# Autodesk Inventor assembly: SACMI DPA TILES GRIP
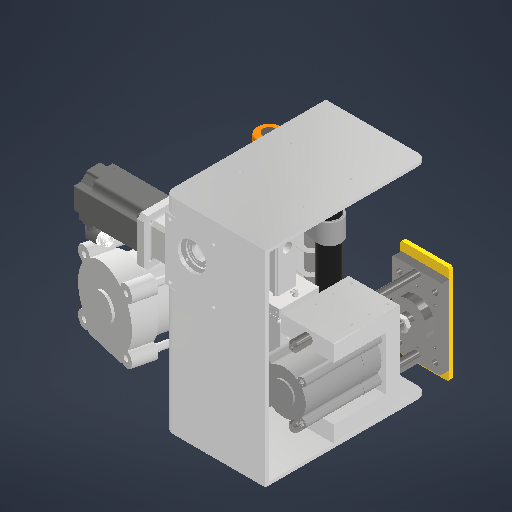
[picture p0: Inventor's stored thumbnail of the model, 512x512]
Saved by Autodesk Inventor 2025 (Build 290162000, 162)
## iProperties
Created: 2024-05-26
Part Number: SACMI DPA TILES GRIP
Document SubType Name: Assembly
Designer: zulet
Author: zulet
## Documents named in this file (7)
- D:\UNAL\2024-1S\APM\Digital Factory\Packaging Machine\SACMI DPA TILES GRIP_MIR.iam
- D:\UNAL\2024-1S\APM\Digital Factory\Linear Guides & Ball Screws\guidage_lineaire_shs55_lv_1_ss___492l_66.iam
- D:\UNAL\2024-1S\APM\Digital Factory\Packaging Machine\Assembly2.iam
- D:\UNAL\2024-1S\APM\Digital Factory\Packaging Machine\TILES GRIP ROLLERS.ipt
- D:\UNAL\2024-1S\APM\Digital Factory\Pneumatic Cylinders and Guides\cylinder_452500010050_010754_0.iam
- D:\UNAL\2024-1S\APM\Digital Factory\Pneumatic Cylinders and Guides\cylinder_45001223510555_0.iam
- D:\UNAL\2024-1S\APM\Digital Factory\Packaging Machine\SACMI DPA TILES GRIP BASE_MIR.ipt
## Components (6 placed, 6 different names)
1. guidage_lineaire_shs55_lv_1_ss___492l_66:1 [sub-assembly] — Rigid:2, Rigid:1
2. Assembly2:1 [sub-assembly] — Cylindrical:3, Mate:1, Angle:1
3. TILES GRIP ROLLERS:1 — Cylindrical:2, Cylindrical:4
4. cylinder_452500010050_010754_0:1 [sub-assembly] — Rigid:1
5. cylinder_45001223510555_0:1 [sub-assembly] — Cylindrical:2, Rotational:2
6. SACMI DPA TILES GRIP BASE_MIR:1 — Cylindrical:3, Mate:1, Angle:1, Rigid:2, Cylindrical:4, Rotational:2
## Relationships (8: CylindricalJoint 3, WeldJoint 2, Mate 1, Angle 1, RevoluteJoint 1)
- Cylindrical:2: TILES GRIP ROLLERS:1 ↔ cylinder_45001223510555_0:1
- Cylindrical:3: Assembly2:1 ↔ SACMI DPA TILES GRIP BASE_MIR:1
- Mate:1: Assembly2:1 ↔ SACMI DPA TILES GRIP BASE_MIR:1
- Angle:1 (0 deg): Assembly2:1 ↔ SACMI DPA TILES GRIP BASE_MIR:1
- Rigid:2 [WeldJoint]: guidage_lineaire_shs55_lv_1_ss___492l_66:1 ↔ SACMI DPA TILES GRIP BASE_MIR:1
- Rigid:1 [WeldJoint]: guidage_lineaire_shs55_lv_1_ss___492l_66:1 ↔ cylinder_452500010050_010754_0:1
- Cylindrical:4: TILES GRIP ROLLERS:1 ↔ SACMI DPA TILES GRIP BASE_MIR:1
- Rotational:2 [RevoluteJoint]: cylinder_45001223510555_0:1 ↔ SACMI DPA TILES GRIP BASE_MIR:1
